# Autodesk Inventor assembly: Assemblage absorbeur
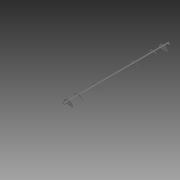
[picture p0: Inventor's stored thumbnail of the model, 180x180]
Saved by Autodesk Inventor 2015 SP1 (Build 190203100, 203)
## iProperties
Created: 2015-05-01
Part Number: Assemblage absorbeur
Document SubType Name: Assembly
Designer: Cyril
Author: Cyril
## Documents named in this file (6)
- C:\Users\Cyril\Documents\OSE FR\Concentrateur solaire\Absorbeur\Assemblage absorbeur.iam
- C:\Users\Cyril\Documents\OSE FR\Concentrateur solaire\Absorbeur\Poutre centrale.ipt
- C:\Users\Cyril\Documents\OSE FR\Concentrateur solaire\Absorbeur\Patron.ipt
- C:\Users\Cyril\Documents\OSE FR\Concentrateur solaire\Absorbeur\Bouchon.ipt
- C:\Users\Cyril\Documents\OSE FR\Concentrateur solaire\Absorbeur\Raccord.ipt
- C:\Users\Cyril\Documents\OSE FR\Concentrateur solaire\Absorbeur\Pied.ipt
## Components (12 placed, 5 different names)
1. Poutre centrale:1 — Mate:1, Mate:2, Mate:3, Mate:4, Mate:9, Mate:10, Angle:1, Mate:11, Mate:12, Mate:13, Mate:14, Mate:15, Mate:16, Mate:17, Mate:18
2. Bouchon:1 — Mate:13, Mate:14
3. Bouchon:2 — Mate:11, Mate:12
4. Raccord:1 — Mate:9, Mate:10, Mate:18
5. Raccord:2 — Mate:15, Mate:16, Mate:17, Mate:19, Mate:20, Mate:21, Mate:22, Mate:23, Mate:24
6. Pied:1 — Mate:19, Mate:20, Mate:21
7. Pied:2 — Mate:22, Mate:23, Mate:24
8. Patron:1 — Mate:3, Mate:4
9. Patron:2
10. Patron:3
11. Patron:4
12. Patron:5
## Component patterns: (5 elements, first: Patron:1)
## Relationships (21: Mate 20, Angle 1)
- Mate:1: Poutre centrale:1
- Mate:2: Poutre centrale:1
- Mate:3: Poutre centrale:1 ↔ Patron:1
- Mate:4: Poutre centrale:1 ↔ Patron:1
- Mate:9: Poutre centrale:1 ↔ Raccord:1
- Mate:10: Poutre centrale:1 ↔ Raccord:1
- Angle:1 (45 deg): Poutre centrale:1
- Mate:11: Poutre centrale:1 ↔ Bouchon:2
- Mate:12: Poutre centrale:1 ↔ Bouchon:2
- Mate:13: Poutre centrale:1 ↔ Bouchon:1
- Mate:14: Poutre centrale:1 ↔ Bouchon:1
- Mate:15: Poutre centrale:1 ↔ Raccord:2
- Mate:16: Poutre centrale:1 ↔ Raccord:2
- Mate:17: Poutre centrale:1 ↔ Raccord:2
- Mate:18: Poutre centrale:1 ↔ Raccord:1
- Mate:19: Raccord:2 ↔ Pied:1
- Mate:20: Raccord:2 ↔ Pied:1
- Mate:21: Raccord:2 ↔ Pied:1
- Mate:22: Raccord:2 ↔ Pied:2
- Mate:23: Raccord:2 ↔ Pied:2
- Mate:24: Raccord:2 ↔ Pied:2
